# Autodesk Inventor assembly: Penholder
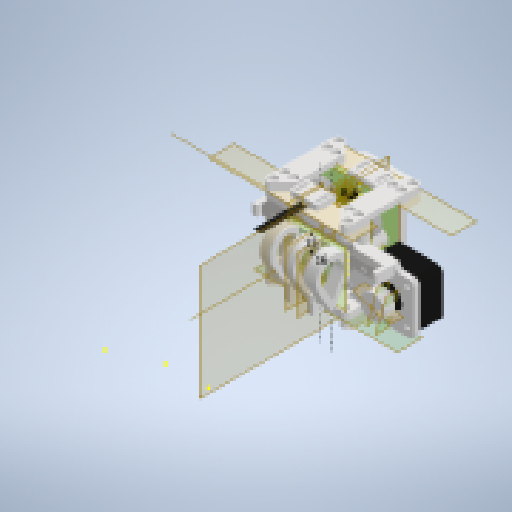
[picture p0: Inventor's stored thumbnail of the model, 512x512]
Saved by Autodesk Inventor 2023 (Build 270158000, 158)
## iProperties
Created: 2023-08-18
Part Number: Penholder
Document SubType Name: Assembly
Designer: Felix
Author: Felix
## Documents named in this file (19)
- D:\Programmieren\PineapplePenPlotter\Inventor\try_3\Penholder.iam
- D:\Programmieren\PineapplePenPlotter\Inventor\try_3\Penholder\Frontside.ipt
- D:\Programmieren\PineapplePenPlotter\Inventor\StoreBought\4022_20220624140806_V-Slot Gantry Kit - 20mm.iam
- D:\Programmieren\PineapplePenPlotter\Inventor\StoreBought\LinearRail.ipt
- D:\Programmieren\PineapplePenPlotter\Inventor\StoreBought\PancakeStepper.ipt
- D:\Programmieren\PineapplePenPlotter\Inventor\try_3\Frontside.ipt
- C:\Users\Felix\Documents\Inventor\Content Center Files\R2023\en-US\DIN EN ISO 4032\DIN EN ISO 4032 - M4.ipt
- C:\Users\Felix\Documents\Inventor\Content Center Files\R2023\en-US\DIN EN ISO 4032\DIN EN ISO 4032 - M5.ipt
- D:\Programmieren\PineapplePenPlotter\Inventor\try_3\StringPulley.ipt
- D:\Programmieren\PineapplePenPlotter\Inventor\StoreBought\LinearRailBlock.ipt
- D:\Programmieren\PineapplePenPlotter\Inventor\try_3\PenHolder.ipt
- D:\Programmieren\PineapplePenPlotter\Inventor\try_3\PenholderPost.ipt
- D:\Programmieren\PineapplePenPlotter\Inventor\try_3\Backside.ipt
- D:\Programmieren\PineapplePenPlotter\Inventor\try_3\GT2BeltSegment.ipt
- D:\Programmieren\PineapplePenPlotter\Inventor\try_3\FixedClamp.ipt
- D:\Programmieren\PineapplePenPlotter\Inventor\try_3\BeltClampNew.ipt
- D:\Programmieren\PineapplePenPlotter\Inventor\try_3\SideBrace.ipt
- D:\Programmieren\PineapplePenPlotter\Inventor\BeltClampM5.ipt
- D:\Programmieren\PineapplePenPlotter\Inventor\SmallBeltClampCover.ipt
## Components (28 placed, 17 different names)
1. Frontside:1
2. 4022_20220624140806_V-Slot Gantry Kit - 20mm:1 [sub-assembly] — Flush:1, Mate:1, Angle:1, Mate:3, Angle:2, Flush:9, Mate:29, Mate:30, Mate:31, Mate:32, Flush:14, Tangent:1, Tangent:2
3. LinearRail:1 — Mate:15, Mate:16, Mate:17, Flush:12, Flush:13
4. PancakeStepper:1 — Mate:18, Flush:34, Mate:27, Mate:28, Angle:5
5. Frontside:2 — Flush:9, Flush:10, Mate:6, Mate:8, Mate:10, Mate:11, Mate:15, Mate:16, Mate:17, Mate:19, Mate:20, Mate:21, Mate:22, Mate:23, Mate:26, Angle:4, Mate:28, Angle:5, Flush:16, Flush:35, Mate:33, Mate:34, Mate:36, Flush:36, Mate:38, Flush:39, Flush:40, Mate:39, Flush:41, Flush:42, Flush:43, Mate:40, Flush:44, Mate:41, Flush:45, Flush:46
6. DIN EN ISO 4032 M4:1 — Mate:6, Mate:20
7. DIN EN ISO 4032 M4:2 — Mate:8, Mate:23
8. DIN EN ISO 4032 M5:1 — Mate:10, Mate:21
9. DIN EN ISO 4032 M5:2 — Mate:11, Mate:22
10. StringPulley:1 — Mate:18, Flush:34
11. LinearRailBlock:1 — Flush:12, Flush:13, Mate:19, Mate:24, Mate:25, Angle:3
12. PenHolder:1 — Mate:24, Mate:25, Angle:3
13. PenholderPost:1 — Mate:29, Mate:30
14. PenholderPost:2 — Mate:31, Mate:32
15. Backside:1 — Flush:15, Flush:16, Flush:36, Flush:37, Mate:37, Tangent:3, Mate:38, Mate:42, Tangent:4
16. GT2BeltSegment:1
17. FixedClamp:2 — Mate:35, Mate:36, Tangent:2
18. FixedClamp:1 — Mate:33, Mate:34, Tangent:1
19. BeltClampNew:1
20. BeltClampNew:2
21. FixedClamp:3 — Mate:37, Tangent:3, Flush:38
22. SideBrace:1 — Flush:39, Flush:40
23. SideBrace:2 — Mate:39, Flush:41, Flush:42
24. SideBrace:3 — Mate:41, Flush:45, Flush:46
25. SideBrace:4 — Flush:43, Mate:40, Flush:44
26. FixedClamp:4 — Mate:42, Tangent:4, Flush:47
27. BeltClampM5:1 — Flush:50
28. SmallBeltClampCover:1 — Flush:50
## Relationships (70: Mate 36, Flush 25, Angle 5, Tangent 4)
- Flush:1 (-11 mm): 4022_20220624140806_V-Slot Gantry Kit - 20mm:1
- Mate:1: 4022_20220624140806_V-Slot Gantry Kit - 20mm:1
- Angle:1 (0 deg): 4022_20220624140806_V-Slot Gantry Kit - 20mm:1
- Flush:5 (3.95 mm)
- Flush:6 (-5.05 mm)
- Mate:3: 4022_20220624140806_V-Slot Gantry Kit - 20mm:1
- Angle:2 (0 deg): 4022_20220624140806_V-Slot Gantry Kit - 20mm:1
- Mate:4
- Mate:5
- Flush:9: 4022_20220624140806_V-Slot Gantry Kit - 20mm:1 ↔ Frontside:2
- Flush:10: Frontside:2
- Mate:6: Frontside:2 ↔ DIN EN ISO 4032 M4:1
- Mate:8: Frontside:2 ↔ DIN EN ISO 4032 M4:2
- Mate:10: Frontside:2 ↔ DIN EN ISO 4032 M5:1
- Mate:11: Frontside:2 ↔ DIN EN ISO 4032 M5:2
- Mate:15: LinearRail:1 ↔ Frontside:2
- Mate:16: LinearRail:1 ↔ Frontside:2
- Mate:17: LinearRail:1 ↔ Frontside:2
- Mate:18: PancakeStepper:1 ↔ StringPulley:1
- Flush:34: PancakeStepper:1 ↔ StringPulley:1
- Flush:12 (2 mm): LinearRail:1 ↔ LinearRailBlock:1
- Flush:13 (-5.5 mm): LinearRail:1 ↔ LinearRailBlock:1
- Mate:19: Frontside:2 ↔ LinearRailBlock:1
- Mate:20: Frontside:2 ↔ DIN EN ISO 4032 M4:1
- Mate:21: Frontside:2 ↔ DIN EN ISO 4032 M5:1
- Mate:22: Frontside:2 ↔ DIN EN ISO 4032 M5:2
- Mate:23: Frontside:2 ↔ DIN EN ISO 4032 M4:2
- Mate:24: LinearRailBlock:1 ↔ PenHolder:1
- Mate:25: LinearRailBlock:1 ↔ PenHolder:1
- Angle:3 (0 deg): LinearRailBlock:1 ↔ PenHolder:1
- Mate:26: Frontside:2
- Angle:4 (0 deg): Frontside:2
- Mate:27: PancakeStepper:1
- Mate:28: PancakeStepper:1 ↔ Frontside:2
- Angle:5 (0 deg): PancakeStepper:1 ↔ Frontside:2
- Mate:29: 4022_20220624140806_V-Slot Gantry Kit - 20mm:1 ↔ PenholderPost:1
- Mate:30: 4022_20220624140806_V-Slot Gantry Kit - 20mm:1 ↔ PenholderPost:1
- Mate:31: 4022_20220624140806_V-Slot Gantry Kit - 20mm:1 ↔ PenholderPost:2
- Mate:32: 4022_20220624140806_V-Slot Gantry Kit - 20mm:1 ↔ PenholderPost:2
- Flush:14 (25 mm): 4022_20220624140806_V-Slot Gantry Kit - 20mm:1
- Flush:15: Backside:1
- Flush:16: Frontside:2 ↔ Backside:1
- Flush:35: Frontside:2
- Mate:33: Frontside:2 ↔ FixedClamp:1
- Mate:34 (1.5 mm): Frontside:2 ↔ FixedClamp:1
- Tangent:1 (1.5 mm): 4022_20220624140806_V-Slot Gantry Kit - 20mm:1 ↔ FixedClamp:1
- Mate:35: FixedClamp:2
- Mate:36 (1.5 mm): Frontside:2 ↔ FixedClamp:2
- Tangent:2 (1.5 mm): 4022_20220624140806_V-Slot Gantry Kit - 20mm:1 ↔ FixedClamp:2
- Flush:36: Frontside:2 ↔ Backside:1
- Flush:37: Backside:1
- Mate:37: Backside:1 ↔ FixedClamp:3
- Tangent:3 (-1.5 mm): Backside:1 ↔ FixedClamp:3
- Flush:38: FixedClamp:3
- Mate:38: Frontside:2 ↔ Backside:1
- Flush:39: Frontside:2 ↔ SideBrace:1
- Flush:40: Frontside:2 ↔ SideBrace:1
- Mate:39: Frontside:2 ↔ SideBrace:2
- Flush:41: Frontside:2 ↔ SideBrace:2
- Flush:42: Frontside:2 ↔ SideBrace:2
- Flush:43: Frontside:2 ↔ SideBrace:4
- Mate:40: Frontside:2 ↔ SideBrace:4
- Flush:44: Frontside:2 ↔ SideBrace:4
- Mate:41: Frontside:2 ↔ SideBrace:3
- Flush:45: Frontside:2 ↔ SideBrace:3
- Flush:46: Frontside:2 ↔ SideBrace:3
- Mate:42: Backside:1 ↔ FixedClamp:4
- Tangent:4 (-1.5 mm): Backside:1 ↔ FixedClamp:4
- Flush:47: FixedClamp:4
- Flush:50: BeltClampM5:1 ↔ SmallBeltClampCover:1
